# Autodesk Inventor assembly: Leg_Frame_Connector_16mm
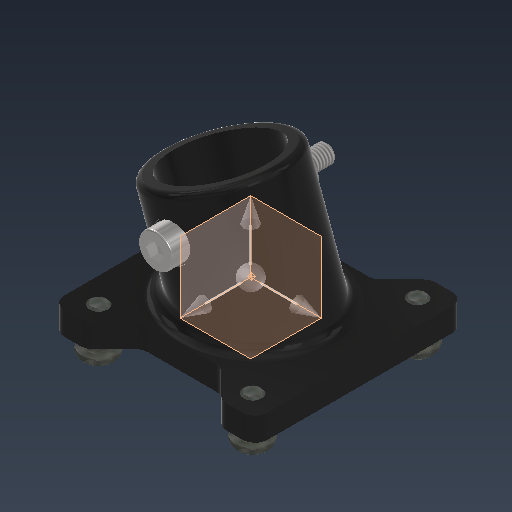
[picture p0: Inventor's stored thumbnail of the model, 512x512]
Saved by Autodesk Inventor 2024.1 (Build 281209000, 209)
## iProperties
Created: 2023-12-05
Part Number: Leg_Frame_Connector_16mm
Document SubType Name: Assembly
Designer: dzw04
Mass: 10.8309 g
Surface Area: 56.3471 cm^2
Volume: 6.63289 cm^3
Density: 1.63291 g/cm^3
Author: dzw04
## Documents named in this file (6)
- C:\Users\dzw04\Saxion\Mechatronica Lectoraat LMECH LED - Database ARG\Component_Database\SARAX\01. CAD\01. 3D_Drawing\02. Sub_Assemblies\Landing_Gear\02. Sub_Assemblies\Leg_Frame_Connector_16mm.iam
- C:\Users\dzw04\Saxion\Mechatronica Lectoraat LMECH LED - Database ARG\Component_Database\SARAX\01. CAD\01. 3D_Drawing\02. Sub_Assemblies\Landing_Gear\01. Parts\Leg_Frame_Connector_16mm.ipt
- C:\Users\dzw04\Saxion\Mechatronica Lectoraat LMECH LED - Database ARG\Component_Database\SARAX\01. CAD\01. 3D_Drawing\01. Parts\en-US\ISO 4762(2)\ISO 4762 - M3 x 25ISO.ipt
- C:\Users\dzw04\Saxion\Mechatronica Lectoraat LMECH LED - Database ARG\Component_Database\SARAX\01. CAD\01. 3D_Drawing\01. Parts\en-US\ISO 4035(2)\ISO 4035 - M3 - ISO.ipt
- C:\Users\dzw04\Saxion\Mechatronica Lectoraat LMECH LED - Database ARG\Component_Database\SARAX\01. CAD\01. 3D_Drawing\01. Parts\en-US\ISO 7380-1\ISO 7380-1 - M3 x 6.ipt
- C:\Users\dzw04\Saxion\Mechatronica Lectoraat LMECH LED - Database ARG\Component_Database\SARAX\01. CAD\01. 3D_Drawing\Parameters.xlsx
## Components (7 placed, 4 different names)
1. Leg_Frame_Connector_16mm:1 — Mate:1, Mate:2, Mate:3, Mate:4, Mate:5, Flush:1, Mate:6, Mate:7, Mate:8
2. ISO 4762 M3 x 25:1 — Mate:1, Mate:2
3. ISO 4035 M3:1 — Mate:3, Mate:4
4. ISO 7380-1 M3 x 6:1 — Mate:7, Mate:8
5. ISO 7380-1 M3 x 6:2
6. ISO 7380-1 M3 x 6:3
7. ISO 7380-1 M3 x 6:4
## Component patterns: (4 elements, first: ISO 7380-1 M3 x 6:1)
## Relationships (9: Mate 8, Flush 1)
- Mate:1: Leg_Frame_Connector_16mm:1 ↔ ISO 4762 M3 x 25:1
- Mate:2: Leg_Frame_Connector_16mm:1 ↔ ISO 4762 M3 x 25:1
- Mate:3: Leg_Frame_Connector_16mm:1 ↔ ISO 4035 M3:1
- Mate:4: Leg_Frame_Connector_16mm:1 ↔ ISO 4035 M3:1
- Mate:5: Leg_Frame_Connector_16mm:1
- Flush:1 (-16.5 mm): Leg_Frame_Connector_16mm:1
- Mate:6 (-17 mm): Leg_Frame_Connector_16mm:1
- Mate:7 (2 mm): Leg_Frame_Connector_16mm:1 ↔ ISO 7380-1 M3 x 6:1
- Mate:8: Leg_Frame_Connector_16mm:1 ↔ ISO 7380-1 M3 x 6:1
## Named parameters: NumberOfArms = 4, RotorToRotor = 900 mm, MountToMotorCenter = 0 mm, ArmPosition = 5 deg, LoadpipeLength = 450 mm, LandingGearHeight = 400 mm, NumberOfBatterys = 2, BatteryLength = 200 mm, BatteryWidth = 62 mm, BatteryHeight = 76 mm, ThicknessBodyOuterPlate = 2 mm, ThicknessBodyCenterPlate = 2 mm, ThicknessLegLoadpipePlate = 2 mm, ThicknessBatteryTray = 2 mm, ThicknessBatteryTopTray = 1 mm, LandingGearRod = 390 mm, LandingGearStabilityBar = 525 mm, StartAngleArm = 45 deg, MotorMountCenter = 71.5 mm
